# Autodesk Inventor assembly: Weather_Station
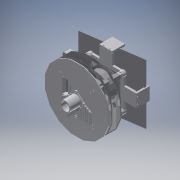
[picture p0: Inventor's stored thumbnail of the model, 180x180]
Saved by Autodesk Inventor 2017 (Build 210142000, 142)
## iProperties
Created: 2019-04-29
Part Number: Weather_Station
Document SubType Name: Assembly
Designer: simulator
Author: simulator
## Documents named in this file (13)
- \\VBOXSVR\Downloads\Weather_Station\Weather_Station.iam
- E:\composite_base.ipt
- E:\boxbase_solar_esp8285.ipt
- E:\cover_clip.ipt
- E:\cone_pattern.ipt
- E:\cover.ipt
- E:\cone_pattern_top2.ipt
- E:\solar roof.ipt
- E:\solar.ipt
- E:\slide_sensor_clip.ipt
- E:\angle_clip.ipt
- E:\side_clip.ipt
- E:\slide_sensor_base.ipt
## Components (13 placed, 12 different names)
1. composite_base:1 — Flush:1, Mate:1, Mate:2, Mate:9, Mate:10, Mate:11
2. boxbase_solar_esp8285:1 — Flush:1, Mate:1, Mate:2, Mate:3, Mate:4, Mate:5, Mate:6, Mate:7, Mate:8
3. cover_clip:1 — Mate:3, Mate:4, Mate:5
4. cone_pattern:1 — Mate:9, Mate:10, Mate:11, Mate:12, Mate:13, Mate:14
5. cover:1 — Mate:6, Mate:7, Mate:8
6. cone_pattern_top2:1 — Mate:12, Mate:13, Mate:14, Mate:15, Mate:16, Mate:17
7. solar roof:1 — Mate:15, Mate:16, Mate:17, Mate:18, Mate:19, Mate:20, Mate:24, Mate:25, Mate:26, Mate:27, Mate:28, Mate:29, Mate:34, Mate:36, Mate:37, Mate:38
8. solar:1 — Mate:33, Mate:34, Mate:35, Mate:39
9. slide_sensor_clip:1 — Mate:27, Mate:28, Mate:29, Mate:30, Mate:31, Mate:32, Mate:35
10. side_clip:1 — Mate:24, Mate:25, Mate:26, Mate:39
11. angle_clip:2 — Mate:18, Mate:19, Mate:20, Mate:33
12. slide_sensor_base:1 — Mate:30, Mate:31, Mate:32
13. side_clip:2 — Mate:36, Mate:37, Mate:38
## Relationships (37: Mate 36, Flush 1)
- Flush:1: composite_base:1 ↔ boxbase_solar_esp8285:1
- Mate:1: composite_base:1 ↔ boxbase_solar_esp8285:1
- Mate:2: composite_base:1 ↔ boxbase_solar_esp8285:1
- Mate:3: boxbase_solar_esp8285:1 ↔ cover_clip:1
- Mate:4: boxbase_solar_esp8285:1 ↔ cover_clip:1
- Mate:5: boxbase_solar_esp8285:1 ↔ cover_clip:1
- Mate:6: boxbase_solar_esp8285:1 ↔ cover:1
- Mate:7: boxbase_solar_esp8285:1 ↔ cover:1
- Mate:8: boxbase_solar_esp8285:1 ↔ cover:1
- Mate:9: composite_base:1 ↔ cone_pattern:1
- Mate:10: composite_base:1 ↔ cone_pattern:1
- Mate:11: composite_base:1 ↔ cone_pattern:1
- Mate:12: cone_pattern:1 ↔ cone_pattern_top2:1
- Mate:13: cone_pattern:1 ↔ cone_pattern_top2:1
- Mate:14: cone_pattern:1 ↔ cone_pattern_top2:1
- Mate:15: cone_pattern_top2:1 ↔ solar roof:1
- Mate:16: cone_pattern_top2:1 ↔ solar roof:1
- Mate:17: cone_pattern_top2:1 ↔ solar roof:1
- Mate:18: solar roof:1 ↔ angle_clip:2
- Mate:19: solar roof:1 ↔ angle_clip:2
- Mate:20: solar roof:1 ↔ angle_clip:2
- Mate:24: solar roof:1 ↔ side_clip:1
- Mate:25: solar roof:1 ↔ side_clip:1
- Mate:26: solar roof:1 ↔ side_clip:1
- Mate:27: solar roof:1 ↔ slide_sensor_clip:1
- Mate:28: solar roof:1 ↔ slide_sensor_clip:1
- Mate:29: solar roof:1 ↔ slide_sensor_clip:1
- Mate:30: slide_sensor_clip:1 ↔ slide_sensor_base:1
- Mate:31: slide_sensor_clip:1 ↔ slide_sensor_base:1
- Mate:32: slide_sensor_clip:1 ↔ slide_sensor_base:1
- Mate:33: solar:1 ↔ angle_clip:2
- Mate:34: solar roof:1 ↔ solar:1
- Mate:35: solar:1 ↔ slide_sensor_clip:1
- Mate:36: solar roof:1 ↔ side_clip:2
- Mate:37: solar roof:1 ↔ side_clip:2
- Mate:38: solar roof:1 ↔ side_clip:2
- Mate:39: solar:1 ↔ side_clip:1
